# Autodesk Inventor assembly: High Strength 60-Tooth Gear-With High Strength Square Gear Insert_MIR6
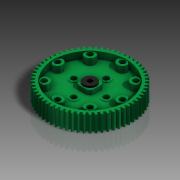
[picture p0: Inventor's stored thumbnail of the model, 180x180]
Saved by Autodesk Inventor 2016 (Build 200138000, 138)
## iProperties
Created: 2010-10-31
Part Number: High Strength 60-Tooth Gear-With High Strength Square Gear Insert_MIR6
Document SubType Name: Assembly
Designer: Afnan
Author: JordanK
## Documents named in this file (3)
- D:\New Laptop\(1) New Laptop\AFNAN ALI flashdrive backup\VEXPARTS\Vex parts\Gears & Pulleys\High Strength 60-Tooth Gear-With High Strength Square Gear Insert_MIR6.iam
- D:\New Laptop\(1) New Laptop\AFNAN ALI flashdrive backup\VEXPARTS\Vex parts\Gears & Pulleys\High Strength 60-Tooth Gear_MIR1.ipt
- D:\New Laptop\(1) New Laptop\AFNAN ALI flashdrive backup\VEXPARTS\Vex parts\Gears & Pulleys\High Strength Square Gear Insert_MIR.ipt
## Components (3 placed, 2 different names)
1. High Strength 60-Tooth Gear_MIR1:1 — Mate:2, Mate:1, Mate:4, Mate:3
2. High Strength Square Gear Insert_MIR:1 — Mate:2, Mate:1
3. High Strength Square Gear Insert_MIR:2 — Mate:4, Mate:3
## Relationships (4: Mate 4)
- Mate:2: High Strength 60-Tooth Gear_MIR1:1 ↔ High Strength Square Gear Insert_MIR:1
- Mate:1: High Strength 60-Tooth Gear_MIR1:1 ↔ High Strength Square Gear Insert_MIR:1
- Mate:4: High Strength 60-Tooth Gear_MIR1:1 ↔ High Strength Square Gear Insert_MIR:2
- Mate:3: High Strength 60-Tooth Gear_MIR1:1 ↔ High Strength Square Gear Insert_MIR:2
